# Autodesk Inventor assembly: stand
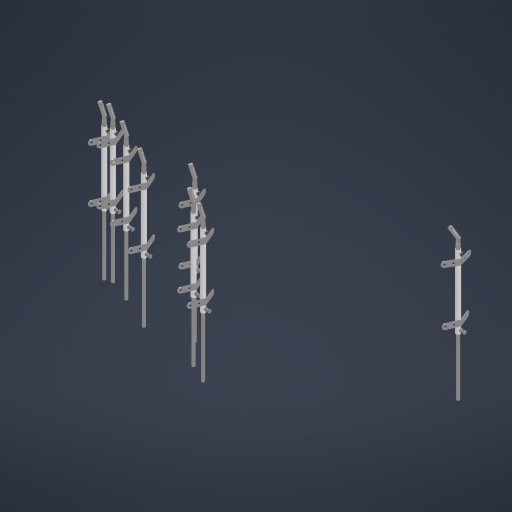
[picture p0: Inventor's stored thumbnail of the model, 512x512]
Saved by Autodesk Inventor 2023 (Build 270158000, 158)
## iProperties
Created: 2022-04-27
Part Number: stand
Document SubType Name: Assembly
Designer: Norbert Ligas
Author: Norbert Ligas
## Documents named in this file (2)
- C:\Users\norbe\Repozytoria\NormalMapScanner\stand_construction\parts\stand.iam
- C:\Users\norbe\Repozytoria\NormalMapScanner\stand_construction\parts\adjustable_leg.iam
## Components (8 placed, 1 different names)
1. adjustable_leg:1 [sub-assembly] — Mate:1, Flush:1, Flush:2, Flush:3
2. adjustable_leg:2 [sub-assembly]
3. adjustable_leg:3 [sub-assembly]
4. adjustable_leg:4 [sub-assembly]
5. adjustable_leg:5 [sub-assembly]
6. adjustable_leg:6 [sub-assembly]
7. adjustable_leg:7 [sub-assembly]
8. adjustable_leg:8 [sub-assembly]
## Relationships (4: Flush 3, Mate 1)
- Mate:1: adjustable_leg:1
- Flush:1: adjustable_leg:1
- Flush:2: adjustable_leg:1
- Flush:3: adjustable_leg:1
